# Autodesk Inventor assembly: ensamble completo
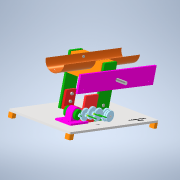
[picture p0: Inventor's stored thumbnail of the model, 180x180]
Saved by Autodesk Inventor 2022 (Build 260153000, 153)
## iProperties
Created: 2022-02-17
Part Number: ensamble completo
Document SubType Name: Assembly
Designer: Home
Author: Home
## Documents named in this file (22)
- C:\Users\Home\Dropbox\2022\DISEÑO E INNOVACIÓN  1\miniproyecto\ensamble completo.iam
- C:\Users\Home\Dropbox\2022\DISEÑO E INNOVACIÓN  1\miniproyecto\base.ipt
- C:\Users\Home\Dropbox\2022\DISEÑO E INNOVACIÓN  1\miniproyecto\angulares.ipt
- C:\Users\Home\Dropbox\2022\DISEÑO E INNOVACIÓN  1\miniproyecto\Columna.ipt
- C:\Users\Home\Dropbox\2022\DISEÑO E INNOVACIÓN  1\miniproyecto\acople_tubo.ipt
- C:\Users\Home\Dropbox\2022\DISEÑO E INNOVACIÓN  1\miniproyecto\tubo PVC.ipt
- C:\Users\Home\Documents\Inventor\Content Center Files\R2022\en-US\ISO 1580\ISO 1580 - M5 x 12_.ipt
- C:\Users\Home\Dropbox\2022\DISEÑO E INNOVACIÓN  1\miniproyecto\eje.ipt
- C:\Users\Home\Dropbox\2022\DISEÑO E INNOVACIÓN  1\miniproyecto\base_motor.ipt
- C:\Users\Home\Documents\Inventor\Content Center Files\R2022\en-US\ISO 1580\ISO 1580 - M5 x 20_.ipt
- C:\Users\Home\Dropbox\2022\DISEÑO E INNOVACIÓN  1\miniproyecto\motor.ipt
- C:\Users\Home\Documents\Inventor\Content Center Files\R2022\en-US\ISO 4032(2)\ISO 4032 - M5 - ISO.ipt
- C:\Users\Home\Documents\Inventor\Content Center Files\R2022\en-US\ISO 1580\ISO 1580 - M5 x 16_.ipt
- C:\Users\Home\Dropbox\2022\DISEÑO E INNOVACIÓN  1\miniproyecto\engrane_motor.ipt
- C:\Users\Home\Dropbox\2022\DISEÑO E INNOVACIÓN  1\miniproyecto\conjunto_engranes.iam
- C:\Users\Home\Dropbox\2022\DISEÑO E INNOVACIÓN  1\miniproyecto\engrane_salida.ipt
- C:\Users\Home\Dropbox\2022\DISEÑO E INNOVACIÓN  1\miniproyecto\eje_salida.ipt
- C:\Users\Home\Dropbox\2022\DISEÑO E INNOVACIÓN  1\miniproyecto\pata_base.ipt
- C:\Users\Home\Dropbox\2022\DISEÑO E INNOVACIÓN  1\miniproyecto\Pared_caja_reduccion.ipt
- C:\Users\Home\Dropbox\2022\DISEÑO E INNOVACIÓN  1\miniproyecto\engrane_32dientes.ipt
- C:\Users\Home\Dropbox\2022\DISEÑO E INNOVACIÓN  1\miniproyecto\Estabilizador.ipt
- C:\Users\Home\Dropbox\2022\DISEÑO E INNOVACIÓN  1\miniproyecto\Pared_caja_reduccion_frontal.ipt
## Components (39 placed, 21 different names)
1. base:1 — Mate:1, Mate:2, Mate:3, Mate:4, Mate:5, Mate:6, Mate:22, Mate:23, Mate:24, Mate:51, Mate:53, Mate:55, Mate:57, Mate:79, Mate:80, Mate:81, Mate:82, Mate:83, Mate:84, Mate:85, Mate:86, Mate:87, Mate:88, Mate:89, Mate:90, Mate:106, Mate:111, Mate:112, Mate:113
2. angulares:1 — Mate:1, Mate:2, Mate:3, Mate:7, Mate:8, Mate:9, Mate:34, Mate:35, Mate:36, Mate:37, Mate:43, Mate:45
3. angulares:2 — Mate:4, Mate:5, Mate:6, Mate:10, Mate:11, Mate:12, Mate:38, Mate:39, Mate:40, Mate:41, Mate:47
4. Columna:1 — Mate:7, Mate:8, Mate:9, Mate:13, Mate:14, Insert:1, Mate:29, Mate:30, Mate:31, Mate:32
5. Columna:2 — Mate:10, Mate:11, Mate:12, Mate:15, Mate:25, Mate:26, Mate:76, Mate:77, Flush:3, Mate:98, Flush:9, Mate:108
6. acople_tubo:1 — Mate:13, Mate:14, Mate:15, Mate:16, Flush:1, Mate:17, Mate:18, Mate:20
7. tubo PVC:1 — Mate:16, Flush:1, Mate:17, Mate:19, Mate:21
8. ISO 1580 M5 x 16:1 — Mate:18, Mate:19
9. ISO 1580 M5 x 12:2 — Mate:20, Mate:21
10. eje:1 — Insert:1, Mate:107
11. base_motor:1 — Mate:22, Mate:23, Mate:24, Mate:33, Flush:8
12. ISO 1580 M5 x 20:1 — Mate:25, Mate:26, Mate:46
13. ISO 1580 M5 x 20:3 — Mate:29, Mate:30, Mate:44
14. ISO 1580 M5 x 20:4 — Mate:31, Mate:32, Mate:42
15. motor:1 — Mate:33, Mate:74, Mate:75, Flush:8
16. ISO 1580 M5 x 20:5 — Mate:34, Mate:35, Mate:56
17. ISO 1580 M5 x 20:6 — Mate:36, Mate:37, Mate:54
18. ISO 1580 M5 x 20:7 — Mate:38, Mate:39, Mate:52
19. ISO 1580 M5 x 20:8 — Mate:40, Mate:41, Mate:50
20. ISO 4032 M5:1 — Mate:42, Mate:43
21. ISO 4032 M5:2 — Mate:44, Mate:45
22. ISO 4032 M5:3 — Mate:46, Mate:47
23. ISO 4032 M5:5 — Mate:50, Mate:51
24. ISO 4032 M5:6 — Mate:52, Mate:53
25. ISO 4032 M5:7 — Mate:54, Mate:55
26. ISO 4032 M5:8 — Mate:56, Mate:57
27. engrane_motor:1 — Mate:74, Mate:75
28. engrane_salida:1 — Mate:76, Flush:7
29. eje_salida:1 — Mate:77, Flush:3
30. pata_base:1 — Mate:79, Mate:80, Mate:81
31. pata_base:2 — Mate:85, Mate:86, Mate:87
32. pata_base:3 — Mate:88, Mate:89, Mate:90
33. pata_base:4 — Mate:82, Mate:83, Mate:84
34. Pared_caja_reduccion:1 — Mate:98, Mate:104, Flush:9, Mate:105, Mate:106, Mate:114, Mate:115, Mate:116
35. engrane_32dientes:1 — Mate:104, Flush:7, Mate:105
36. Estabilizador:1 — Mate:107, Mate:108
37. Pared_caja_reduccion_frontal:1 — Mate:111, Mate:112, Mate:113
38. conjunto_engranes:1 [sub-assembly] — Mate:114, Mate:117
39. conjunto_engranes:2 [sub-assembly] — Mate:115, Mate:116, Mate:117
## Relationships (88: Mate 82, Flush 5, Insert 1)
- Mate:1: base:1 ↔ angulares:1
- Mate:2: base:1 ↔ angulares:1
- Mate:3: base:1 ↔ angulares:1
- Mate:4: base:1 ↔ angulares:2
- Mate:5: base:1 ↔ angulares:2
- Mate:6: base:1 ↔ angulares:2
- Mate:7: angulares:1 ↔ Columna:1
- Mate:8: angulares:1 ↔ Columna:1
- Mate:9: angulares:1 ↔ Columna:1
- Mate:10: angulares:2 ↔ Columna:2
- Mate:11: angulares:2 ↔ Columna:2
- Mate:12: angulares:2 ↔ Columna:2
- Mate:13: Columna:1 ↔ acople_tubo:1
- Mate:14 (2 mm): Columna:1 ↔ acople_tubo:1
- Mate:15: Columna:2 ↔ acople_tubo:1
- Mate:16: acople_tubo:1 ↔ tubo PVC:1
- Flush:1: acople_tubo:1 ↔ tubo PVC:1
- Mate:17: acople_tubo:1 ↔ tubo PVC:1
- Mate:18: acople_tubo:1 ↔ ISO 1580 M5 x 16:1
- Mate:19: tubo PVC:1 ↔ ISO 1580 M5 x 16:1
- Mate:20: acople_tubo:1 ↔ ISO 1580 M5 x 12:2
- Mate:21: tubo PVC:1 ↔ ISO 1580 M5 x 12:2
- Insert:1 (-7 mm): Columna:1 ↔ eje:1
- Mate:22: base:1 ↔ base_motor:1
- Mate:23: base:1 ↔ base_motor:1
- Mate:24: base:1 ↔ base_motor:1
- Mate:25: Columna:2 ↔ ISO 1580 M5 x 20:1
- Mate:26: Columna:2 ↔ ISO 1580 M5 x 20:1
- Mate:29: Columna:1 ↔ ISO 1580 M5 x 20:3
- Mate:30: Columna:1 ↔ ISO 1580 M5 x 20:3
- Mate:31: Columna:1 ↔ ISO 1580 M5 x 20:4
- Mate:32: Columna:1 ↔ ISO 1580 M5 x 20:4
- Mate:33: base_motor:1 ↔ motor:1
- Mate:34: angulares:1 ↔ ISO 1580 M5 x 20:5
- Mate:35: angulares:1 ↔ ISO 1580 M5 x 20:5
- Mate:36: angulares:1 ↔ ISO 1580 M5 x 20:6
- Mate:37: angulares:1 ↔ ISO 1580 M5 x 20:6
- Mate:38: angulares:2 ↔ ISO 1580 M5 x 20:7
- Mate:39: angulares:2 ↔ ISO 1580 M5 x 20:7
- Mate:40: angulares:2 ↔ ISO 1580 M5 x 20:8
- Mate:41: angulares:2 ↔ ISO 1580 M5 x 20:8
- Mate:42: ISO 1580 M5 x 20:4 ↔ ISO 4032 M5:1
- Mate:43: angulares:1 ↔ ISO 4032 M5:1
- Mate:44: ISO 1580 M5 x 20:3 ↔ ISO 4032 M5:2
- Mate:45: angulares:1 ↔ ISO 4032 M5:2
- Mate:46: ISO 1580 M5 x 20:1 ↔ ISO 4032 M5:3
- Mate:47: angulares:2 ↔ ISO 4032 M5:3
- Mate:50: ISO 1580 M5 x 20:8 ↔ ISO 4032 M5:5
- Mate:51: base:1 ↔ ISO 4032 M5:5
- Mate:52: ISO 1580 M5 x 20:7 ↔ ISO 4032 M5:6
- Mate:53: base:1 ↔ ISO 4032 M5:6
- Mate:54: ISO 1580 M5 x 20:6 ↔ ISO 4032 M5:7
- Mate:55: base:1 ↔ ISO 4032 M5:7
- Mate:56: ISO 1580 M5 x 20:5 ↔ ISO 4032 M5:8
- Mate:57: base:1 ↔ ISO 4032 M5:8
- Mate:74: motor:1 ↔ engrane_motor:1
- Mate:75 (1 mm): motor:1 ↔ engrane_motor:1
- Mate:76: Columna:2 ↔ engrane_salida:1
- Mate:77: Columna:2 ↔ eje_salida:1
- Flush:3 (-30 mm): Columna:2 ↔ eje_salida:1
- Mate:79: base:1 ↔ pata_base:1
- Mate:80: base:1 ↔ pata_base:1
- Mate:81: base:1 ↔ pata_base:1
- Mate:82: base:1 ↔ pata_base:4
- Mate:83: base:1 ↔ pata_base:4
- Mate:84: base:1 ↔ pata_base:4
- Mate:85: base:1 ↔ pata_base:2
- Mate:86: base:1 ↔ pata_base:2
- Mate:87: base:1 ↔ pata_base:2
- Mate:88: base:1 ↔ pata_base:3
- Mate:89: base:1 ↔ pata_base:3
- Mate:90: base:1 ↔ pata_base:3
- Mate:98: Columna:2 ↔ Pared_caja_reduccion:1
- Mate:104: Pared_caja_reduccion:1 ↔ engrane_32dientes:1
- Flush:7: engrane_salida:1 ↔ engrane_32dientes:1
- Flush:8 (-7.5 mm): base_motor:1 ↔ motor:1
- Flush:9: Columna:2 ↔ Pared_caja_reduccion:1
- Mate:105: Pared_caja_reduccion:1 ↔ engrane_32dientes:1
- Mate:106: base:1 ↔ Pared_caja_reduccion:1
- Mate:107: eje:1 ↔ Estabilizador:1
- Mate:108 (21.6 mm): Columna:2 ↔ Estabilizador:1
- Mate:111: base:1 ↔ Pared_caja_reduccion_frontal:1
- Mate:112: base:1 ↔ Pared_caja_reduccion_frontal:1
- Mate:113: base:1 ↔ Pared_caja_reduccion_frontal:1
- Mate:114: Pared_caja_reduccion:1 ↔ conjunto_engranes:1
- Mate:115: Pared_caja_reduccion:1 ↔ conjunto_engranes:2
- Mate:116 (0.5 mm): Pared_caja_reduccion:1 ↔ conjunto_engranes:2
- Mate:117 (0.12 mm): conjunto_engranes:1 ↔ conjunto_engranes:2
